# Autodesk Inventor assembly: Beam
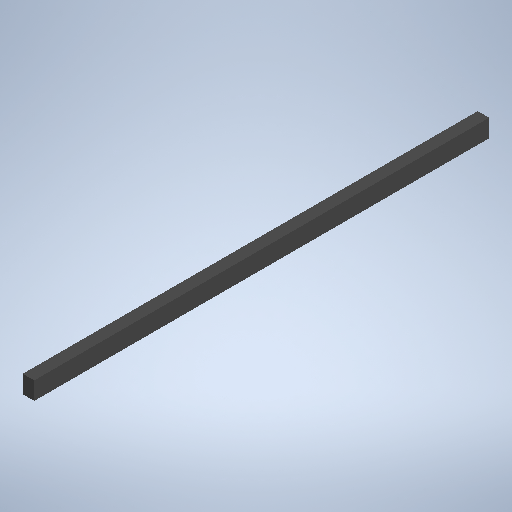
[picture p0: Inventor's stored thumbnail of the model, 512x512]
Saved by Autodesk Inventor 2025 (Build 290162010, 162A)
## iProperties
Created: 2024-09-15
Part Number: Beam
Document SubType Name: Assembly
Designer: Tom
Author: Tom
## Documents named in this file (4)
- C:\Users\Tom\Documents\Inventor\Mobility\Additional_Building\Beam.iam
- C:\Users\Tom\Documents\Inventor\Mobility\Additional_Building\Beam.ipt
- C:\Users\Tom\Documents\Inventor\Mobility\Additional_Building\Rectangle_Of_Underlayment_For_Beam.ipt
- C:\Users\Tom\Documents\Inventor\Mobility\Additional_Building\Tube_Of_Underlayment_For_Beam.ipt
## Components (4 placed, 3 different names)
1. Beam:1 — Mate:1, Flush:1, Flush:2, Mate:2, Flush:3, Flush:4, Mate:3, Mate:4
2. Rectangle_Of_Underlayment_For_Beam:1 — Mate:1, Flush:1, Flush:2, Flush:5
3. Rectangle_Of_Underlayment_For_Beam:2 — Mate:2, Flush:3, Flush:4
4. Tube_Of_Underlayment_For_Beam:1 — Mate:3, Mate:4, Flush:5
## Relationships (9: Flush 5, Mate 4)
- Mate:1: Beam:1 ↔ Rectangle_Of_Underlayment_For_Beam:1
- Flush:1: Beam:1 ↔ Rectangle_Of_Underlayment_For_Beam:1
- Flush:2: Beam:1 ↔ Rectangle_Of_Underlayment_For_Beam:1
- Mate:2: Beam:1 ↔ Rectangle_Of_Underlayment_For_Beam:2
- Flush:3: Beam:1 ↔ Rectangle_Of_Underlayment_For_Beam:2
- Flush:4: Beam:1 ↔ Rectangle_Of_Underlayment_For_Beam:2
- Mate:3: Beam:1 ↔ Tube_Of_Underlayment_For_Beam:1
- Mate:4: Beam:1 ↔ Tube_Of_Underlayment_For_Beam:1
- Flush:5: Rectangle_Of_Underlayment_For_Beam:1 ↔ Tube_Of_Underlayment_For_Beam:1
